# Autodesk Inventor assembly: CannonV2
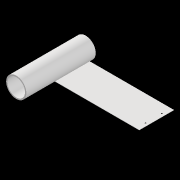
[picture p0: Inventor's stored thumbnail of the model, 180x180]
Saved by Autodesk Inventor 2022 (Build 260153000, 153)
## iProperties
Created: 2021-10-10
Part Number: CannonV2
Document SubType Name: Assembly
Designer: timmy
Author: timmy
## Documents named in this file (3)
- S:\Inventor\RoboCatz\T-Shirt\CannonV2.iam
- S:\Inventor\RoboCatz\T-Shirt\cannonplate.ipt
- S:\Inventor\RoboCatz\T-Shirt\3FT-SCH40-PVC.ipt
## Components (2 placed, 2 different names)
1. cannonplate:1 — Flush:1, Tangent:1
2. 3FT-SCH40-PVC:1 — Flush:1, Tangent:1
## Relationships (2: Flush 1, Tangent 1)
- Flush:1: cannonplate:1 ↔ 3FT-SCH40-PVC:1
- Tangent:1: cannonplate:1 ↔ 3FT-SCH40-PVC:1
